# Autodesk Inventor assembly: servo_mount_assembly
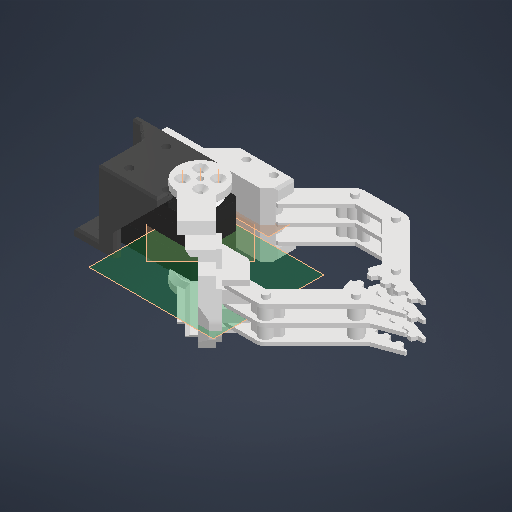
[picture p0: Inventor's stored thumbnail of the model, 512x512]
Saved by Autodesk Inventor 2026 (Build 300175000, 175)
## iProperties
Created: 2025-03-27
Part Number: servo_mount_assembly
Document SubType Name: Assembly
Designer: paris
Author: paris
## Documents named in this file (6)
- C:\Users\paris\OneDrive\Documents\GitHub\and-e\robot_manipulator_cad_files\Workspaces\Workspace\servo_mount_assembly.iam
- C:\Users\paris\OneDrive\Documents\GitHub\and-e\robot_manipulator_cad_files\Workspaces\Workspace\custom_servo_bracket.ipt
- C:\Users\paris\OneDrive\Documents\GitHub\and-e\robot_manipulator_cad_files\Workspaces\Workspace\ST3215.iam
- C:\Users\paris\OneDrive\Documents\GitHub\and-e\robot_manipulator_cad_files\Workspaces\Workspace\claw_dynamic_gripper_assembly.iam
- C:\Users\paris\OneDrive\Documents\GitHub\and-e\robot_manipulator_cad_files\Workspaces\Workspace\claw_static_gripper_assembly.iam
- C:\Users\paris\OneDrive\Documents\GitHub\and-e\robot_manipulator_cad_files\Workspaces\Workspace\new_custom_servo_claw_bracket.ipt
## Components (5 placed, 5 different names)
1. custom_servo_bracket:1 — Mate:1, Mate:2, Mate:3, Mate:6, Mate:7, Mate:8
2. ST3215:1 [sub-assembly] — Mate:1, Mate:2, Mate:3, Flush:1
3. claw_dynamic_gripper_assembly:1 [sub-assembly]
4. claw_static_gripper_assembly:1 [sub-assembly] — Mate:6, Mate:7, Mate:8
5. new_custom_servo_claw_bracket:1 — Flush:1
## Relationships (7: Mate 6, Flush 1)
- Mate:1: custom_servo_bracket:1 ↔ ST3215:1
- Mate:2: custom_servo_bracket:1 ↔ ST3215:1
- Mate:3: custom_servo_bracket:1 ↔ ST3215:1
- Mate:6: custom_servo_bracket:1 ↔ claw_static_gripper_assembly:1
- Mate:7: custom_servo_bracket:1 ↔ claw_static_gripper_assembly:1
- Mate:8: custom_servo_bracket:1 ↔ claw_static_gripper_assembly:1
- Flush:1: ST3215:1 ↔ new_custom_servo_claw_bracket:1
